# Autodesk Inventor assembly: A2017_T4_05
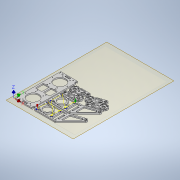
[picture p0: Inventor's stored thumbnail of the model, 180x180]
Saved by Autodesk Inventor 2020 (Build 240168000, 168)
## iProperties
Created: 2021-08-27
Part Number: A2017_T4_05
Document SubType Name: Assembly
Designer: Masato
Author: Masato
## Documents named in this file (5)
- C:\Users\aibay\Documents\Inventor\cam\sustaina\SUSTAINA-OP\Cam\A2017_T4_05.iam
- C:\Users\aibay\Documents\Inventor\cam\sustaina\SUSTAINA-OP\Cam\DisposableBoard.ipt
- C:\Users\aibay\Documents\Inventor\cam\sustaina\SUSTAINA-OP\UpperBody\Trunk\Trunk_shoulder_frame.ipt
- C:\Users\aibay\Documents\Inventor\cam\sustaina\SUSTAINA-OP\UpperBody\Trunk\Trunk_waisit_frame.ipt
- C:\Users\aibay\Documents\Inventor\cam\sustaina\SUSTAINA-OP\LowerBody\Ankle\Ankle_side_pitch_frame.ipt
## Components (8 placed, 4 different names)
1. DisposableBoard:1 — メイト:2, メイト:1, フラッシュ:1, フラッシュ:2, メイト:4, メイト:5, メイト:6, メイト:7, メイト:8, フラッシュ:3, フラッシュ:4, メイト:15, メイト:16
2. Trunk_shoulder_frame:1 — メイト:4, メイト:10, メイト:11, 正接:1, メイト:17, メイト:18, 正接:4
3. Trunk_shoulder_frame:2 — メイト:5, フラッシュ:5, メイト:9, メイト:11
4. Trunk_waisit_frame:1 — メイト:6, フラッシュ:3, フラッシュ:4, フラッシュ:5, メイト:9, メイト:10, 正接:2, 正接:3
5. Ankle_side_pitch_frame:1 — メイト:8, メイト:14, 正接:3
6. Ankle_side_pitch_frame:2 — メイト:7, メイト:14, 正接:1, メイト:17, 正接:2, 正接:5
7. Ankle_side_pitch_frame:3 — メイト:16, メイト:19, 正接:5
8. Ankle_side_pitch_frame:4 — メイト:15, メイト:18, 正接:4, メイト:19
## Relationships (26: Mate 16, Flush 5, Tangent 5)
- メイト:2 [Mate]: DisposableBoard:1
- メイト:1 [Mate]: DisposableBoard:1
- フラッシュ:1 [Flush]: DisposableBoard:1
- フラッシュ:2 [Flush]: DisposableBoard:1
- メイト:4 [Mate]: DisposableBoard:1 ↔ Trunk_shoulder_frame:1
- メイト:5 [Mate]: DisposableBoard:1 ↔ Trunk_shoulder_frame:2
- メイト:6 [Mate]: DisposableBoard:1 ↔ Trunk_waisit_frame:1
- メイト:7 [Mate]: DisposableBoard:1 ↔ Ankle_side_pitch_frame:2
- メイト:8 [Mate]: DisposableBoard:1 ↔ Ankle_side_pitch_frame:1
- フラッシュ:3 [Flush] (2 mm): DisposableBoard:1 ↔ Trunk_waisit_frame:1
- フラッシュ:4 [Flush] (2 mm): DisposableBoard:1 ↔ Trunk_waisit_frame:1
- フラッシュ:5 [Flush]: Trunk_shoulder_frame:2 ↔ Trunk_waisit_frame:1
- メイト:9 [Mate] (2.5 mm): Trunk_shoulder_frame:2 ↔ Trunk_waisit_frame:1
- メイト:10 [Mate] (2.5 mm): Trunk_shoulder_frame:1 ↔ Trunk_waisit_frame:1
- メイト:11 [Mate] (2.5 mm): Trunk_shoulder_frame:1 ↔ Trunk_shoulder_frame:2
- メイト:14 [Mate] (2.5 mm): Ankle_side_pitch_frame:1 ↔ Ankle_side_pitch_frame:2
- 正接:1 [Tangent] (2.5 mm): Trunk_shoulder_frame:1 ↔ Ankle_side_pitch_frame:2
- メイト:15 [Mate]: DisposableBoard:1 ↔ Ankle_side_pitch_frame:4
- メイト:16 [Mate]: DisposableBoard:1 ↔ Ankle_side_pitch_frame:3
- メイト:17 [Mate] (2.5 mm): Trunk_shoulder_frame:1 ↔ Ankle_side_pitch_frame:2
- 正接:2 [Tangent] (2.5 mm): Trunk_waisit_frame:1 ↔ Ankle_side_pitch_frame:2
- 正接:3 [Tangent] (2.5 mm): Trunk_waisit_frame:1 ↔ Ankle_side_pitch_frame:1
- メイト:18 [Mate] (2.5 mm): Trunk_shoulder_frame:1 ↔ Ankle_side_pitch_frame:4
- 正接:4 [Tangent] (5 mm): Trunk_shoulder_frame:1 ↔ Ankle_side_pitch_frame:4
- メイト:19 [Mate] (2.5 mm): Ankle_side_pitch_frame:3 ↔ Ankle_side_pitch_frame:4
- 正接:5 [Tangent] (2.5 mm): Ankle_side_pitch_frame:2 ↔ Ankle_side_pitch_frame:3
